# Autodesk Inventor assembly: xy-motion-asm
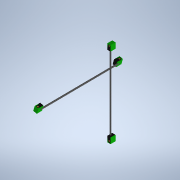
[picture p0: Inventor's stored thumbnail of the model, 180x180]
Saved by Autodesk Inventor 2020.4 (Build 244396000, 396)
## iProperties
Created: 2021-03-31
Part Number: xy-motion-asm
Document SubType Name: Assembly
Designer: AOB
Mass: 170.12 g
Surface Area: 811.196 cm^2
Volume: 70.9394 cm^3
Density: 2.39811 g/cm^3
Author: AOB
## Documents named in this file (4)
- C:\Users\marti\Documents\Inventor\ProjectBoron\Boron Ultima\xy-motion-asm.iam
- C:\Users\marti\Documents\Inventor\ProjectBoron\Boron Ultima\Y-linear bearing shroud.iam
- C:\Users\marti\Documents\Inventor\ProjectBoron\Boron Ultima\X-linear bearing shroud.iam
- C:\Users\marti\Documents\Inventor\ProjectBoron\Boron Ultima\8mm carbon fiber rod.ipt
## Components (6 placed, 3 different names)
1. Y-linear bearing shroud:1 [sub-assembly] — Rigid:3
2. Y-linear bearing shroud:2 [sub-assembly] — Rigid:4
3. X-linear bearing shroud:1 [sub-assembly] — Rigid:1
4. X-linear bearing shroud:2 [sub-assembly] — Rigid:2
5. 8mm carbon fiber rod:1 — Rigid:1, Rigid:2, Angle:1
6. 8mm carbon fiber rod:2 — Rigid:3, Rigid:4, Angle:1
## Relationships (5: WeldJoint 4, Angle 1)
- Rigid:1 [WeldJoint]: X-linear bearing shroud:1 ↔ 8mm carbon fiber rod:1
- Rigid:2 [WeldJoint]: X-linear bearing shroud:2 ↔ 8mm carbon fiber rod:1
- Rigid:3 [WeldJoint] (-9.5399 mm): Y-linear bearing shroud:1 ↔ 8mm carbon fiber rod:2
- Rigid:4 [WeldJoint] (9.5399 mm): Y-linear bearing shroud:2 ↔ 8mm carbon fiber rod:2
- Angle:1 (90 deg): 8mm carbon fiber rod:1 ↔ 8mm carbon fiber rod:2
